# Autodesk Inventor assembly: BRACKET_ASSEMBLY
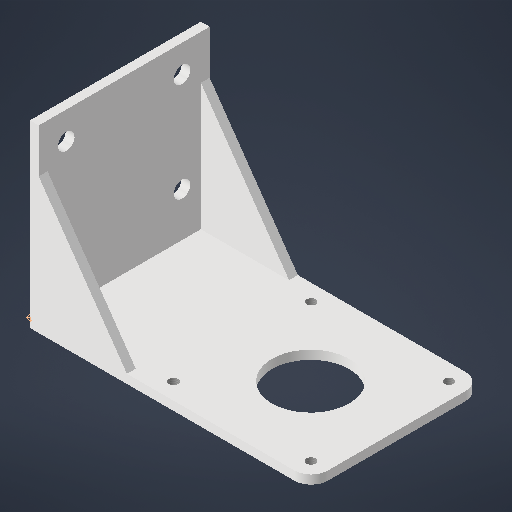
[picture p0: Inventor's stored thumbnail of the model, 512x512]
Saved by Autodesk Inventor 2026.1 (Build 301233020, 233B)
## iProperties
Created: 2025-10-11
Part Number: BRACKET_ASSEMBLY
Document SubType Name: Weldment
Designer: Alexander
Weld Material: Welded Aluminum-6061
Author: Alexander
## Documents named in this file (4)
- C:\Users\Alexander\Documents\M&M Engineering Second year\Semester 2\Introductory Machine Design 254\Theory of Machines\Project\Part 2\BRACKET_ASSEMBLY.iam
- C:\Users\Alexander\Documents\M&M Engineering Second year\Semester 2\Introductory Machine Design 254\Theory of Machines\Project\Part 2\BRACKET BASE.ipt
- C:\Users\Alexander\Documents\M&M Engineering Second year\Semester 2\Introductory Machine Design 254\Theory of Machines\Project\Part 2\Bracket_side.ipt
- C:\Users\Alexander\Documents\M&M Engineering Second year\Semester 2\Introductory Machine Design 254\Theory of Machines\Project\Part 2\BRACKET GUSSET.ipt
## Components (4 placed, 3 different names)
1. BRACKET BASE:1 — Mate:1, Mate:2, Mate:3, Mate:5
2. Bracket_side:1 — Mate:1, Mate:2, Mate:4, Mate:6, Mate:7
3. BRACKET GUSSET:1 — Mate:3, Mate:4
4. BRACKET GUSSET:2 — Mate:5, Mate:6
## Relationships (7: Mate 7)
- Mate:1: BRACKET BASE:1 ↔ Bracket_side:1
- Mate:2: BRACKET BASE:1 ↔ Bracket_side:1
- Mate:3: BRACKET BASE:1 ↔ BRACKET GUSSET:1
- Mate:4: Bracket_side:1 ↔ BRACKET GUSSET:1
- Mate:5: BRACKET BASE:1 ↔ BRACKET GUSSET:2
- Mate:6: Bracket_side:1 ↔ BRACKET GUSSET:2
- Mate:7: Bracket_side:1
